# Autodesk Inventor assembly: mascon-new
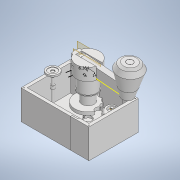
[picture p0: Inventor's stored thumbnail of the model, 180x180]
Saved by Autodesk Inventor 2021 (Build 250183000, 183)
## iProperties
Created: 2021-04-28
Part Number: mascon-new
Document SubType Name: Assembly
Designer: ben
Author: ben
## Documents named in this file (12)
- C:\Users\teh18\OneDrive\BVE Controller\r68-bve-mascon\mascon-new.iam
- C:\Users\teh18\OneDrive\BVE Controller\r68-bve-mascon\handle-base\handle-base.iam
- C:\Users\teh18\OneDrive\BVE Controller\r68-bve-mascon\handle\handle.iam
- C:\Users\teh18\OneDrive\BVE Controller\r68-bve-mascon\shell\shell.iam
- C:\Users\teh18\OneDrive\BVE Controller\r68-bve-mascon\handle_base2.ipt
- C:\Users\teh18\OneDrive\BVE Controller\r68-bve-mascon\handle_base3.ipt
- C:\Users\teh18\OneDrive\BVE Controller\r68-bve-mascon\handle_base_rod.ipt
- C:\Users\teh18\OneDrive\BVE Controller\r68-bve-mascon\handle_base_potholder.ipt
- C:\Users\teh18\OneDrive\BVE Controller\r68-bve-mascon\handle_holder.ipt
- C:\Users\teh18\OneDrive\BVE Controller\r68-bve-mascon\Reverser.ipt
- C:\Users\teh18\OneDrive\BVE Controller\r68-bve-mascon\reverser-base.ipt
- C:\Users\teh18\OneDrive\BVE Controller\r68-bve-mascon\NotchClickerAsm.iam
## Components (11 placed, 11 different names)
1. handle-base:1 [sub-assembly] — handle pop, Mate:3, Mate:4, Mate:5, Mate:6, Mate:8, Flush:3, Mate:9, Mate:10
2. handle:1 [sub-assembly] — handle pop
3. shell:1 [sub-assembly] — Mate:3, Flush:4, Mate:10, Mate:12
4. handle_base2:1 — Mate:4, Flush:1, Mate:5, Mate:6, Mate:11
5. handle_base3:1 — Flush:1, Flush:2
6. handle_base_rod:1 — Mate:8, Mate:11
7. handle_base_potholder:1 — Flush:2
8. handle_holder:1 — Flush:3, Mate:9
9. Reverser:1 — Flush:4, Flush:5
10. reverser-base:1 — Flush:5
11. NotchClickerAsm:1 [sub-assembly] — Mate:12
## Relationships (15: Mate 9, Flush 5, RevoluteJoint 1)
- handle pop [RevoluteJoint]: handle-base:1 ↔ handle:1
- Mate:3: handle-base:1 ↔ shell:1
- Mate:4: handle-base:1 ↔ handle_base2:1
- Flush:1: handle_base2:1 ↔ handle_base3:1
- Mate:5: handle-base:1 ↔ handle_base2:1
- Mate:6: handle-base:1 ↔ handle_base2:1
- Mate:8: handle-base:1 ↔ handle_base_rod:1
- Flush:2: handle_base3:1 ↔ handle_base_potholder:1
- Flush:3: handle-base:1 ↔ handle_holder:1
- Mate:9: handle-base:1 ↔ handle_holder:1
- Flush:4: shell:1 ↔ Reverser:1
- Flush:5: Reverser:1 ↔ reverser-base:1
- Mate:10: handle-base:1 ↔ shell:1
- Mate:11: handle_base2:1 ↔ handle_base_rod:1
- Mate:12: shell:1 ↔ NotchClickerAsm:1
